# Autodesk Inventor assembly: Assembly2
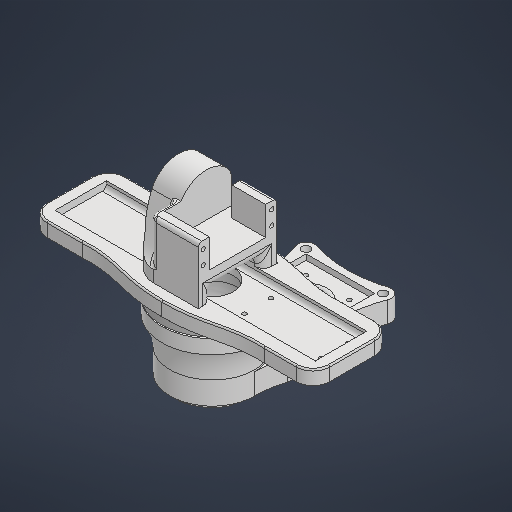
[picture p0: Inventor's stored thumbnail of the model, 512x512]
Saved by Autodesk Inventor 2026.1 (Build 301233020, 233B)
## iProperties
Created: 2025-10-29
Part Number: Assembly2
Document SubType Name: Assembly
Designer: Piter
Author: Piter
## Documents named in this file (4)
- C:\Users\Piotrek\Desktop\Robots\David\Davie-Robot-Arm\3D Models\Assembly2.iam
- C:\Users\Piotrek\Desktop\Robots\David\Davie-Robot-Arm\3D Models\Base_top.ipt
- C:\Users\Piotrek\Desktop\Robots\David\Davie-Robot-Arm\3D Models\axis_shaft.ipt
- C:\Users\Piotrek\Desktop\Robots\David\Davie-Robot-Arm\3D Models\Axis1_top.ipt
## Components (3 placed, 3 different names)
1. Base_top:1 — Rotational:1
2. axis_shaft:1 — Rotational:1, Rigid:1
3. Axis1_top:1 — Rigid:1
## Relationships (2: RevoluteJoint 1, WeldJoint 1)
- Rotational:1 [RevoluteJoint] (-1 mm): Base_top:1 ↔ axis_shaft:1
- Rigid:1 [WeldJoint]: axis_shaft:1 ↔ Axis1_top:1
